# Autodesk Inventor assembly: U_SECTION
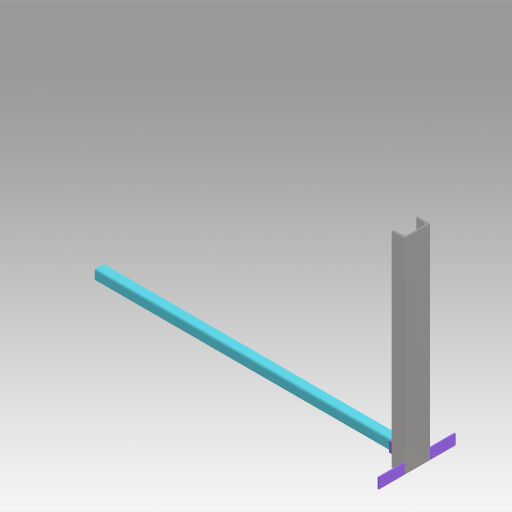
[picture p0: Inventor's stored thumbnail of the model, 512x512]
Saved by Autodesk Inventor 2023 (Build 270158000, 158)
## iProperties
_SolveAssemblyDoc: Frame Generator Solve Assembly
_Version: 15.0.0
Created: 2025-04-08
Part Number: U_SECTION
Document SubType Name: Assembly
Designer: NELLY NDUNG'U
Author: NELLY NDUNG'U
## Documents named in this file (5)
- N:\NAKUJA\CAD FILES\AIRFRAME\LP002\U_SECTION.iam
- N:\NAKUJA\CAD FILES\AIRFRAME\LP002\U_SECTION.ipt
- N:\NAKUJA\CAD FILES\AIRFRAME\LP002\U_SECTION\Frame\Frame 1744091750735.iam
- N:\NAKUJA\CAD FILES\AIRFRAME\LP002\LEG_ATTACHMENT.ipt
- N:\NAKUJA\CAD FILES\AIRFRAME\LP002\LEG.iam
## Components (6 placed, 4 different names)
1. U_SECTION:1
2. Frame 1744091750735:1 [sub-assembly] — Flush:1, Mate:1, Flush:2, Mate:2, Flush:3, Flush:4, Mate:3, Flush:5, Mate:4, Mate:6
3. LEG_ATTACHMENT:1 — Flush:1, Mate:1, Flush:2
4. LEG_ATTACHMENT:2 — Mate:2, Flush:3, Flush:4
5. LEG_ATTACHMENT:3 — Mate:3, Flush:5, Mate:4, Mate:5, Flush:6
6. LEG:1 [sub-assembly] — Mate:5, Flush:6, Mate:6
## Relationships (12: Flush 6, Mate 6)
- Flush:1: Frame 1744091750735:1 ↔ LEG_ATTACHMENT:1
- Mate:1: Frame 1744091750735:1 ↔ LEG_ATTACHMENT:1
- Flush:2: Frame 1744091750735:1 ↔ LEG_ATTACHMENT:1
- Mate:2: Frame 1744091750735:1 ↔ LEG_ATTACHMENT:2
- Flush:3: Frame 1744091750735:1 ↔ LEG_ATTACHMENT:2
- Flush:4: Frame 1744091750735:1 ↔ LEG_ATTACHMENT:2
- Mate:3: Frame 1744091750735:1 ↔ LEG_ATTACHMENT:3
- Flush:5: Frame 1744091750735:1 ↔ LEG_ATTACHMENT:3
- Mate:4 (50 mm): Frame 1744091750735:1 ↔ LEG_ATTACHMENT:3
- Mate:5: LEG_ATTACHMENT:3 ↔ LEG:1
- Flush:6: LEG_ATTACHMENT:3 ↔ LEG:1
- Mate:6 (5 mm): Frame 1744091750735:1 ↔ LEG:1
